# Autodesk Inventor assembly: 000-3p-robot-v4
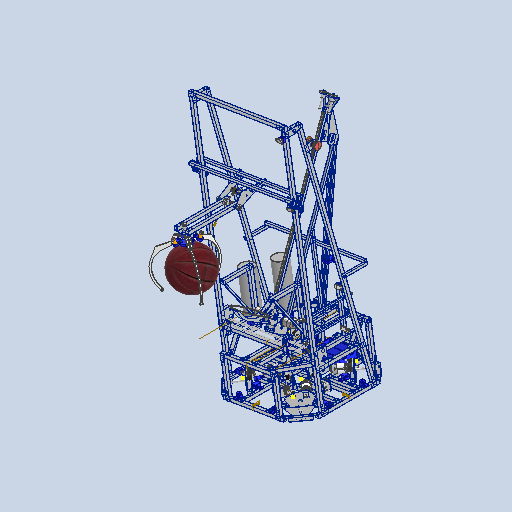
[picture p0: Inventor's stored thumbnail of the model, 512x512]
Saved by Autodesk Inventor 2025.2 (Build 292293000, 293)
## iProperties
Created: 2025-04-03
Part Number: 000-3p-robot-v4
Document SubType Name: Assembly
Designer: haruy
Author: haruy
## Documents named in this file (4)
- C:\Users\haruy\Documents\ロボコン\NHK2025\cad\nagahisa\000-3p-robot-v4.iam
- C:\Users\haruy\Documents\ロボコン\NHK2025\cad\nagahisa\base_weel\000-base_wheel-v3.iam
- C:\Users\haruy\Documents\ロボコン\NHK2025\cad\nagahisa\dribl\000-dribl-v2.iam
- C:\Users\haruy\Documents\ロボコン\NHK2025\cad\nagahisa\belt_liner\000-belt_liner_v5.iam
## Components (3 placed, 3 different names)
1. 000-base_wheel-v3:1 [sub-assembly] — フラッシュ:1, メイト:1, フラッシュ:2
2. 000-dribl-v2:1 [sub-assembly] — フラッシュ:1, メイト:1, フラッシュ:2, 挿入:1, 挿入:2
3. 000-belt_liner_v5:1 [sub-assembly] — 挿入:1, 挿入:2
## Relationships (5: Flush 2, Insert 2, Mate 1)
- フラッシュ:1 [Flush]: 000-base_wheel-v3:1 ↔ 000-dribl-v2:1
- メイト:1 [Mate]: 000-base_wheel-v3:1 ↔ 000-dribl-v2:1
- フラッシュ:2 [Flush] (20 mm): 000-base_wheel-v3:1 ↔ 000-dribl-v2:1
- 挿入:1 [Insert]: 000-dribl-v2:1 ↔ 000-belt_liner_v5:1
- 挿入:2 [Insert]: 000-dribl-v2:1 ↔ 000-belt_liner_v5:1
